# Autodesk Inventor assembly: Grant's gargantuanly gregariously garish gearbox
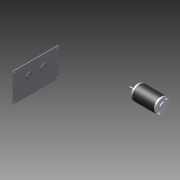
[picture p0: Inventor's stored thumbnail of the model, 180x180]
Saved by Autodesk Inventor 2015 (Build 190159000, 159)
## iProperties
Created: 2015-01-28
Part Number: Grant's gargantuanly gregariously garish gearbox
Document SubType Name: Assembly
Designer: whitaus15
Author: whitaus15
## Documents named in this file (13)
- \\lhssvr02\Homedirs\Robotics Club\CAD Model 2015\Grant\Grant's gargantuanly gregariously garish gearbox.iam
- \\lhssvr02\Homedirs\Robotics Club\CAD Model 2015\Grant\gear.ipt
- \\lhssvr02\Homedirs\Robotics Club\CAD Model 2015\Grant\Sprocket Large.ipt
- \\lhssvr02\Homedirs\Robotics Club\CAD Model 2015\Grant\Gearbox plate.ipt
- \\lhssvr02\Homedirs\Robotics Club\CAD Model 2015\Grant\MOT_CIM-Motor_217-2000.iam.iam
- \\lhssvr02\Homedirs\Robotics Club\CAD Model 2015\Box Beam Drive Base\Newest\Hex Shaft for E gear box.ipt
- \\lhssvr02\Homedirs\Robotics Club\CAD Model 2015\Box Beam Drive Base\brf-08.ipt
- \\lhssvr02\Homedirs\Robotics Club\CAD Model 2015\Grant\gear_MIR2.ipt
- \\lhssvr02\Homedirs\Robotics Club\CAD Model 2015\Grant\Sprocket Large_MIR2.ipt
- \\lhssvr02\Homedirs\Robotics Club\CAD Model 2015\Box Beam Drive Base\Newest\Hex Shaft for E gear box_MIR2.ipt
- \\lhssvr02\Homedirs\Robotics Club\CAD Model 2015\Box Beam Drive Base\brf-08_MIR.ipt
- \\lhssvr02\Homedirs\Robotics Club\CAD Model 2015\Grant\Gearbox plate with motor.ipt
- MOT_CIM-Motor_217-2000.iam
## Components (13 placed, 11 different names)
1. gear:2 — Mate:44, Mate:45, Mate:47, Mate:54
2. Sprocket Large:1 — Mate:46, Mate:47, Mate:48
3. Gearbox plate:2 — Mate:29, Mate:33, Angle:1, Insert:1, Insert:5
4. MOT_CIM-Motor_217-2000.iam:1 [sub-assembly] — Angle:1
5. Hex Shaft for E gear box:1 — Mate:44, Mate:45, Mate:46, Mate:48, Tangent:1, Insert:3, Insert:9
6. brf-08:1 — Insert:1, Tangent:1, Insert:3, Mate:54
7. gear_MIR2:1 — Mate:55, Mate:58, Mate:59, Mate:60
8. Sprocket Large_MIR2:1 — Mate:55, Mate:56, Mate:57
9. Hex Shaft for E gear box_MIR2:1 — Mate:56, Mate:57, Mate:58, Mate:59, Insert:4, Tangent:2, Insert:8
10. brf-08_MIR:1 — Mate:60, Insert:4, Tangent:2, Insert:5
11. Gearbox plate with motor:1 — Insert:6, Insert:7
12. brf-08:2 — Insert:7, Insert:9
13. brf-08:3 — Insert:6, Insert:8
## Relationships (26: Mate 15, Insert 8, Tangent 2, Angle 1)
- Mate:16
- Mate:29: Gearbox plate:2
- Mate:33: Gearbox plate:2
- Angle:1 (0 deg): Gearbox plate:2 ↔ MOT_CIM-Motor_217-2000.iam:1
- Mate:44: gear:2 ↔ Hex Shaft for E gear box:1
- Mate:45: gear:2 ↔ Hex Shaft for E gear box:1
- Mate:46: Sprocket Large:1 ↔ Hex Shaft for E gear box:1
- Mate:47: gear:2 ↔ Sprocket Large:1
- Mate:48: Sprocket Large:1 ↔ Hex Shaft for E gear box:1
- Insert:1: Gearbox plate:2 ↔ brf-08:1
- Tangent:1: Hex Shaft for E gear box:1 ↔ brf-08:1
- Insert:3: Hex Shaft for E gear box:1 ↔ brf-08:1
- Mate:54: gear:2 ↔ brf-08:1
- Mate:55: gear_MIR2:1 ↔ Sprocket Large_MIR2:1
- Mate:56: Sprocket Large_MIR2:1 ↔ Hex Shaft for E gear box_MIR2:1
- Mate:57: Sprocket Large_MIR2:1 ↔ Hex Shaft for E gear box_MIR2:1
- Mate:58: gear_MIR2:1 ↔ Hex Shaft for E gear box_MIR2:1
- Mate:59: gear_MIR2:1 ↔ Hex Shaft for E gear box_MIR2:1
- Mate:60: gear_MIR2:1 ↔ brf-08_MIR:1
- Insert:4: Hex Shaft for E gear box_MIR2:1 ↔ brf-08_MIR:1
- Tangent:2: Hex Shaft for E gear box_MIR2:1 ↔ brf-08_MIR:1
- Insert:5: Gearbox plate:2 ↔ brf-08_MIR:1
- Insert:6: Gearbox plate with motor:1 ↔ brf-08:3
- Insert:7: Gearbox plate with motor:1 ↔ brf-08:2
- Insert:8: Hex Shaft for E gear box_MIR2:1 ↔ brf-08:3
- Insert:9: Hex Shaft for E gear box:1 ↔ brf-08:2
